# Autodesk Inventor assembly: BDR_Full Extension Ball bearing Slide1
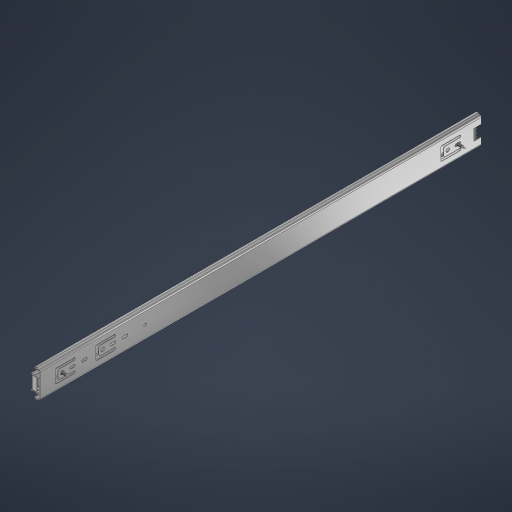
[picture p0: Inventor's stored thumbnail of the model, 512x512]
Saved by Autodesk Inventor 2024.3 (Build 283343000, 343)
## iProperties
Created: 2013-11-19
Part Number: BDR_Full Extension Ball bearing Slide1
Document SubType Name: Assembly
Designer: SauliusD
Description: Full Extension Ball bearing Slide
Author: SauliusD
## Documents named in this file (6)
- C:\W4INV 2024 Design\PROJECTS\Living Room\Bed\Drawer\BDR_Full Extension Ball bearing Slide1.iam
- C:\W4INV 2024 Design\PROJECTS\Samples\Living Room\Bed\Drawer\BDR_Outer Slider Guide1.ipt
- C:\W4INV 2024 Design\PROJECTS\Samples\Living Room\Bed\Drawer\BDR_Secondary Slider Guide1.ipt
- C:\W4INV 2024 Design\PROJECTS\Samples\Living Room\Bed\Drawer\BDR_Inner Slider Guide1.ipt
- C:\W4INV 2024 Design\PROJECTS\Samples\Living Room\Bed\Drawer\BDR_Bumper1.ipt
- C:\W4INV 2024 Design\PROJECTS\Samples\Living Room\Bed\Drawer\BDR_Screw 11.ipt
## Components (8 placed, 5 different names)
1. BDR_Outer Slider Guide1:1 — Insert:2, Mate:1, Mate:2
2. BDR_Secondary Slider Guide1:1
3. BDR_Inner Slider Guide1:1 — Insert:1
4. BDR_Bumper1:1
5. BDR_Screw 11:1
6. BDR_Screw 11:2 — Insert:1
7. BDR_Screw 11:3 — Insert:2
8. BDR_Screw 11:4 — Mate:1, Mate:2
## Relationships (4: Insert 2, Mate 2)
- Insert:1: BDR_Inner Slider Guide1:1 ↔ BDR_Screw 11:2
- Insert:2: BDR_Outer Slider Guide1:1 ↔ BDR_Screw 11:3
- Mate:1: BDR_Outer Slider Guide1:1 ↔ BDR_Screw 11:4
- Mate:2: BDR_Outer Slider Guide1:1 ↔ BDR_Screw 11:4
